# Autodesk Inventor assembly: Dock
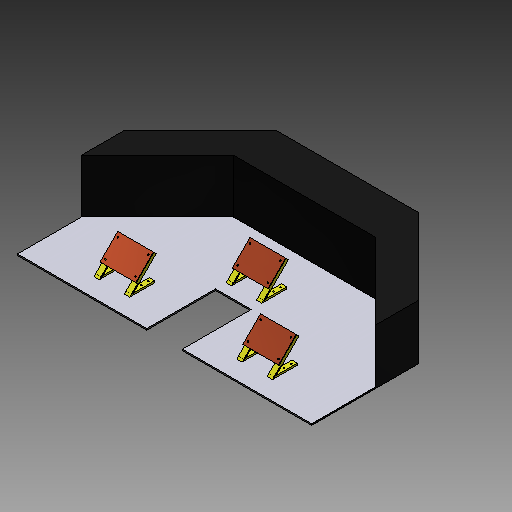
[picture p0: Inventor's stored thumbnail of the model, 512x512]
Saved by Autodesk Inventor 2018 (Build 220112000, 112)
## iProperties
Created: 2017-06-02
Part Number: Dock
Document SubType Name: Assembly
Designer: AYUSH SHUKLA
Author: AYUSH SHUKLA
## Documents named in this file (4)
- C:\Study\BTP2\Robomuse Inventor CAD\Dock\Dock.iam
- C:\Study\BTP2\Robomuse Inventor CAD\Dock\Dock_Base.ipt
- C:\Study\BTP2\Robomuse Inventor CAD\Dock\pedal.ipt
- C:\Study\BTP2\Robomuse Inventor CAD\Dock\Copper_Plate.ipt
## Components (10 placed, 3 different names)
1. Dock_Base:1 — Mate:1, Mate:2, Mate:3, Mate:4, Mate:5, Mate:6, Mate:7, Mate:8, Mate:9, Mate:10, Mate:11, Mate:12, Mate:13, Mate:14, Mate:15, Mate:16, Mate:17, Mate:18
2. pedal:1 — Mate:4, Mate:9, Mate:10, Mate:19, Mate:21
3. pedal:2 — Mate:5, Mate:13, Mate:14, Mate:23
4. pedal:3 — Mate:6, Mate:11, Mate:12, Mate:20, Mate:24
5. pedal:4 — Mate:7, Mate:15, Mate:16, Flush:1
6. pedal:5 — Mate:8, Mate:17, Mate:18
7. pedal:6 — Mate:1, Mate:2, Mate:3, Mate:22
8. Copper_Plate:1 — Flush:1
9. Copper_Plate:2 — Mate:19, Mate:21, Mate:22
10. Copper_Plate:3 — Mate:20, Mate:23, Mate:24
## Relationships (25: Mate 24, Flush 1)
- Mate:1: Dock_Base:1 ↔ pedal:6
- Mate:2: Dock_Base:1 ↔ pedal:6
- Mate:3: Dock_Base:1 ↔ pedal:6
- Mate:4: Dock_Base:1 ↔ pedal:1
- Mate:5: Dock_Base:1 ↔ pedal:2
- Mate:6: Dock_Base:1 ↔ pedal:3
- Mate:7: Dock_Base:1 ↔ pedal:4
- Mate:8: Dock_Base:1 ↔ pedal:5
- Mate:9: Dock_Base:1 ↔ pedal:1
- Mate:10: Dock_Base:1 ↔ pedal:1
- Mate:11: Dock_Base:1 ↔ pedal:3
- Mate:12: Dock_Base:1 ↔ pedal:3
- Mate:13: Dock_Base:1 ↔ pedal:2
- Mate:14: Dock_Base:1 ↔ pedal:2
- Mate:15: Dock_Base:1 ↔ pedal:4
- Mate:16: Dock_Base:1 ↔ pedal:4
- Mate:17: Dock_Base:1 ↔ pedal:5
- Mate:18: Dock_Base:1 ↔ pedal:5
- Flush:1: pedal:4 ↔ Copper_Plate:1
- Mate:19: pedal:1 ↔ Copper_Plate:2
- Mate:20: pedal:3 ↔ Copper_Plate:3
- Mate:21: pedal:1 ↔ Copper_Plate:2
- Mate:22: pedal:6 ↔ Copper_Plate:2
- Mate:23: pedal:2 ↔ Copper_Plate:3
- Mate:24: pedal:3 ↔ Copper_Plate:3
